# Autodesk Inventor assembly: Ensamblaje1
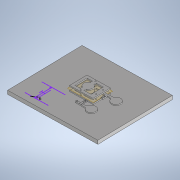
[picture p0: Inventor's stored thumbnail of the model, 180x180]
Saved by Autodesk Inventor 2022 (Build 260153000, 153)
## iProperties
Created: 2022-11-13
Part Number: Ensamblaje1
Document SubType Name: Assembly
Designer: Usuario
Author: Usuario
## Documents named in this file (6)
- C:\Users\Usuario\Documents\Cosas de Sebastian\Robotica\PROYECTO\CAD\GRIPPER\Ensamblaje1.iam
- C:\Users\Usuario\Documents\Cosas de Sebastian\Robotica\PROYECTO\CAD\GRIPPER\BASE.ipt
- C:\Users\Usuario\Documents\Cosas de Sebastian\Robotica\PROYECTO\CAD\GRIPPER\BASE_UP.ipt
- C:\Users\Usuario\Documents\Cosas de Sebastian\Robotica\PROYECTO\CAD\GRIPPER\PINZA_D.ipt
- C:\Users\Usuario\Documents\Cosas de Sebastian\Robotica\PROYECTO\CAD\GRIPPER\PINZA_I.ipt
- C:\Users\Usuario\Documents\Cosas de Sebastian\Robotica\PROYECTO\CAD\GRIPPER\Placa.ipt
## Components (5 placed, 5 different names)
1. BASE:1 — Rígido:1, Rígido:2
2. BASE_UP:1 — Rígido:2
3. PINZA_D:1 — De rotación:1, Ángulo:1
4. PINZA_I:1
5. Placa:1 — Rígido:1, De rotación:1, Ángulo:1
## Relationships (4: WeldJoint 2, RevoluteJoint 1, Angle 1)
- Rígido:1 [WeldJoint]: BASE:1 ↔ Placa:1
- Rígido:2 [WeldJoint]: BASE:1 ↔ BASE_UP:1
- De rotación:1 [RevoluteJoint] (-13 mm): PINZA_D:1 ↔ Placa:1
- Ángulo:1 [Angle] (0 deg): PINZA_D:1 ↔ Placa:1
